# Autodesk Inventor assembly: Złożenie
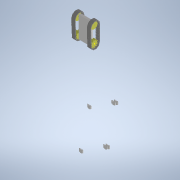
[picture p0: Inventor's stored thumbnail of the model, 180x180]
Saved by Autodesk Inventor 2022 (Build 260153000, 153)
## iProperties
Created: 2022-04-03
Part Number: Złożenie
Document SubType Name: Assembly
Designer: jolow
Author: jolow
## Documents named in this file (6)
- E:\Modele inventor\SR\PROJEKTZESPOLOWY\Złożenie.iam
- E:\Modele inventor\SR\PROJEKTZESPOLOWY\pudelko dol.ipt
- E:\Modele inventor\SR\PROJEKTZESPOLOWY\KOŁO.ipt
- E:\Modele inventor\SR\PROJEKTZESPOLOWY\Silniczek.ipt
- E:\Modele inventor\SR\PROJEKTZESPOLOWY\gasienica.ipt
- E:\Modele inventor\SR\PROJEKTZESPOLOWY\Koło napinające.ipt
## Components (53 placed, 5 different names)
1. pudelko dol:1 — Zestawiające:1, Zestawiające:2, Zestawiające:3, Zestawiające:4, Zestawiające:5, Zestawiające:22
2. KOŁO:1 — Zestawiające:6, Zestawiające:7
3. KOŁO:2 — Zestawiające:8, Zestawiające:9
4. Silniczek:1 — Zestawiające:1, Zestawiające:2, Zestawiające:8, Zestawiające:9
5. Silniczek:2 — Zestawiające:3, Zestawiające:4, Zestawiające:5, Zestawiające:6, Zestawiające:7
6. gasienica:1 — Zestawiające:10, Zestawiające:11, Zestawiające:12, Zestawiające:13
7. gasienica:2 — Zestawiające:10, Zestawiające:11, Zestawiające:18, Zestawiające:19
8. gasienica:3 — Zestawiające:12, Zestawiające:13, Zestawiające:14, Zestawiające:15
9. gasienica:4 — Zestawiające:14, Zestawiające:15, Zestawiające:16, Zestawiające:17
10. gasienica:5 — Zestawiające:16, Zestawiające:17, Zestawiające:51
11. gasienica:7 — Zestawiające:18, Zestawiające:19, Zestawiające:23, Zestawiające:24
12. gasienica:10 — Zestawiające:27, Zestawiające:28, Zestawiające:29, Zestawiające:30
13. gasienica:11 — Zestawiające:29, Zestawiające:30, Zestawiające:31, Zestawiające:32
14. gasienica:13 — Zestawiające:25, Zestawiające:26, Zestawiające:27, Zestawiające:28
15. gasienica:14 — Zestawiające:23, Zestawiające:24, Zestawiające:25, Zestawiające:26
16. Koło napinające:1 — Zestawiające:22
17. gasienica:15 — Zestawiające:37, Zestawiające:38, Zestawiające:39, Zestawiające:40
18. gasienica:17 — Zestawiające:47, Zestawiające:48, Zestawiające:49, Zestawiające:50
19. gasienica:18 — Zestawiające:31, Zestawiające:32, Zestawiające:33, Zestawiające:34
20. gasienica:19
21. gasienica:20 — Zestawiające:42, Zestawiające:44, Zestawiające:45, Zestawiające:46
22. gasienica:21 — Zestawiające:39, Zestawiające:40, Zestawiające:41, Zestawiające:43
23. gasienica:22 — Zestawiające:41, Zestawiające:42, Zestawiające:43, Zestawiające:44
24. gasienica:23 — Zestawiające:45, Zestawiające:46, Zestawiające:47, Zestawiające:48
25. gasienica:24 — Zestawiające:49, Zestawiające:50, Zestawiające:51
26. gasienica:25 — Zestawiające:33, Zestawiające:34, Zestawiające:35, Zestawiające:36
27. gasienica:26
28. gasienica:27
29. gasienica:28 — Zestawiające:35, Zestawiające:36, Zestawiające:37, Zestawiające:38
30. gasienica:29
31. gasienica:30
32. gasienica:31
33. gasienica:32
34. gasienica:33
35. gasienica:34
36. gasienica:35
37. gasienica:36
38. gasienica:37
39. gasienica:38
40. Koło napinające:2
41. gasienica:39
42. gasienica:40
43. gasienica:41
44. gasienica:42
45. gasienica:43
46. gasienica:44
47. gasienica:45
48. gasienica:46
49. gasienica:47
50. gasienica:48
51. gasienica:49
52. gasienica:50
53. gasienica:51
## Relationships (88: Mate 88)
- Zestawiające:1 [Mate]: pudelko dol:1 ↔ Silniczek:1
- Zestawiające:2 [Mate]: pudelko dol:1 ↔ Silniczek:1
- Zestawiające:3 [Mate]: pudelko dol:1 ↔ Silniczek:2
- Zestawiające:4 [Mate]: pudelko dol:1 ↔ Silniczek:2
- Zestawiające:5 [Mate]: pudelko dol:1 ↔ Silniczek:2
- Zestawiające:6 [Mate]: KOŁO:1 ↔ Silniczek:2
- Zestawiające:7 [Mate]: KOŁO:1 ↔ Silniczek:2
- Zestawiające:8 [Mate]: KOŁO:2 ↔ Silniczek:1
- Zestawiające:9 [Mate]: KOŁO:2 ↔ Silniczek:1
- Zestawiające:10 [Mate]: gasienica:1 ↔ gasienica:2
- Zestawiające:11 [Mate]: gasienica:1 ↔ gasienica:2
- Zestawiające:12 [Mate]: gasienica:1 ↔ gasienica:3
- Zestawiające:13 [Mate]: gasienica:1 ↔ gasienica:3
- Zestawiające:14 [Mate]: gasienica:3 ↔ gasienica:4
- Zestawiające:15 [Mate]: gasienica:3 ↔ gasienica:4
- Zestawiające:16 [Mate]: gasienica:4 ↔ gasienica:5
- Zestawiające:17 [Mate]: gasienica:4 ↔ gasienica:5
- Zestawiające:18 [Mate]: gasienica:2 ↔ gasienica:7
- Zestawiające:19 [Mate]: gasienica:2 ↔ gasienica:7
- Zestawiające:22 [Mate]: pudelko dol:1 ↔ Koło napinające:1
- Zestawiające:23 [Mate]: gasienica:7 ↔ gasienica:14
- Zestawiające:24 [Mate]: gasienica:7 ↔ gasienica:14
- Zestawiające:25 [Mate]: gasienica:13 ↔ gasienica:14
- Zestawiające:26 [Mate]: gasienica:13 ↔ gasienica:14
- Zestawiające:27 [Mate]: gasienica:10 ↔ gasienica:13
- Zestawiające:28 [Mate]: gasienica:10 ↔ gasienica:13
- Zestawiające:29 [Mate]: gasienica:10 ↔ gasienica:11
- Zestawiające:30 [Mate]: gasienica:10 ↔ gasienica:11
- Zestawiające:31 [Mate]: gasienica:11 ↔ gasienica:18
- Zestawiające:32 [Mate]: gasienica:11 ↔ gasienica:18
- Zestawiające:33 [Mate]: gasienica:18 ↔ gasienica:25
- Zestawiające:34 [Mate]: gasienica:18 ↔ gasienica:25
- Zestawiające:35 [Mate]: gasienica:25 ↔ gasienica:28
- Zestawiające:36 [Mate]: gasienica:25 ↔ gasienica:28
- Zestawiające:37 [Mate]: gasienica:15 ↔ gasienica:28
- Zestawiające:38 [Mate]: gasienica:15 ↔ gasienica:28
- Zestawiające:39 [Mate]: gasienica:15 ↔ gasienica:21
- Zestawiające:40 [Mate]: gasienica:15 ↔ gasienica:21
- Zestawiające:41 [Mate]: gasienica:21 ↔ gasienica:22
- Zestawiające:42 [Mate]: gasienica:20 ↔ gasienica:22
- Zestawiające:43 [Mate]: gasienica:21 ↔ gasienica:22
- Zestawiające:44 [Mate]: gasienica:20 ↔ gasienica:22
- Zestawiające:45 [Mate]: gasienica:20 ↔ gasienica:23
- Zestawiające:46 [Mate]: gasienica:20 ↔ gasienica:23
- Zestawiające:47 [Mate]: gasienica:17 ↔ gasienica:23
- Zestawiające:48 [Mate]: gasienica:17 ↔ gasienica:23
- Zestawiające:49 [Mate]: gasienica:17 ↔ gasienica:24
- Zestawiające:50 [Mate]: gasienica:17 ↔ gasienica:24
- Zestawiające:51 [Mate]: gasienica:5 ↔ gasienica:24
- [Mate]: gasienica:29 ↔ gasienica:30
- [Mate]: gasienica:29 ↔ gasienica:30
- [Mate]: gasienica:29 ↔ gasienica:31
- [Mate]: gasienica:29 ↔ gasienica:31
- [Mate]: gasienica:31 ↔ gasienica:32
- [Mate]: gasienica:31 ↔ gasienica:32
- [Mate]: gasienica:32 ↔ gasienica:33
- [Mate]: gasienica:32 ↔ gasienica:33
- [Mate]: gasienica:30 ↔ gasienica:34
- [Mate]: gasienica:30 ↔ gasienica:34
- [Mate]: gasienica:34 ↔ gasienica:38
- [Mate]: gasienica:34 ↔ gasienica:38
- [Mate]: gasienica:37 ↔ gasienica:38
- [Mate]: gasienica:37 ↔ gasienica:38
- [Mate]: gasienica:35 ↔ gasienica:37
- [Mate]: gasienica:35 ↔ gasienica:37
- [Mate]: gasienica:35 ↔ gasienica:36
- [Mate]: gasienica:35 ↔ gasienica:36
- [Mate]: gasienica:36 ↔ gasienica:41
- [Mate]: gasienica:36 ↔ gasienica:41
- [Mate]: gasienica:41 ↔ gasienica:48
- [Mate]: gasienica:41 ↔ gasienica:48
- [Mate]: gasienica:48 ↔ gasienica:51
- [Mate]: gasienica:48 ↔ gasienica:51
- [Mate]: gasienica:39 ↔ gasienica:51
- [Mate]: gasienica:39 ↔ gasienica:51
- [Mate]: gasienica:39 ↔ gasienica:44
- [Mate]: gasienica:39 ↔ gasienica:44
- [Mate]: gasienica:44 ↔ gasienica:45
- [Mate]: gasienica:43 ↔ gasienica:45
- [Mate]: gasienica:44 ↔ gasienica:45
- [Mate]: gasienica:43 ↔ gasienica:45
- [Mate]: gasienica:43 ↔ gasienica:46
- [Mate]: gasienica:43 ↔ gasienica:46
- [Mate]: gasienica:40 ↔ gasienica:46
- [Mate]: gasienica:40 ↔ gasienica:46
- [Mate]: gasienica:40 ↔ gasienica:47
- [Mate]: gasienica:40 ↔ gasienica:47
- [Mate]: gasienica:33 ↔ gasienica:47
## Named parameters: d59_d35 = 0 mm, d60_d36 = 0 mm, d61_d37 = 0 mm, d62_d38 = 0 mm, d63_d39 = 0 mm, d64_d40 = 0 mm, d65_d41 = 0 mm, d66_d42 = 0 mm, d67_d43 = 0 mm, d68_d44 = 0 mm, d69_d45 = 0 mm, d70_d46 = 0 mm, d71_d47 = 0 mm, d72_d48 = 0 mm, d73_d49 = 0 mm, d74_d50 = 0 mm, d75_d51 = 0 mm, d76_d52 = 0 mm, d77_d53 = 0 mm, d78_d58 = 0 mm, d79_d9 = 0 mm, d80_d10 = 0 mm, d81_d11 = 0 mm, d82_d12 = 0 mm, d83_d13 = 0 mm, d84_d14 = 0 mm, d85_d15 = 0 mm, d86_d16 = 0 mm, d87_d17 = 0 mm, d88_d18 = 0 mm, d89_d26 = 0 mm, d90_d27 = 0 mm, d91_d28 = 0 mm, d92_d29 = 0 mm, d93_d30 = 0 mm, d94_d31 = 0 mm, d95_d32 = 0 mm, d96_d33 = 0 mm, d97_d34 = 0 mm
